# Autodesk Inventor assembly: Telemetry TAZ V1
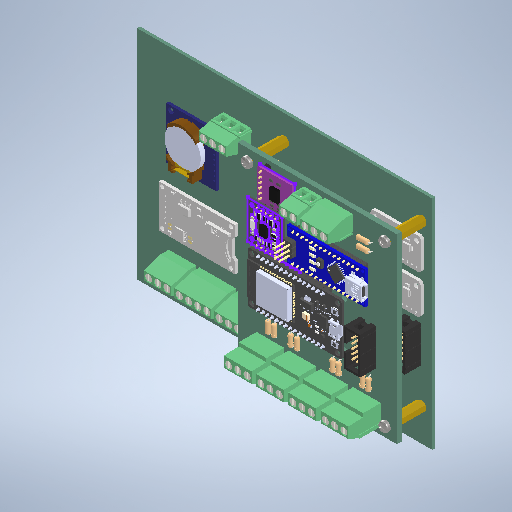
[picture p0: Inventor's stored thumbnail of the model, 512x512]
Saved by Autodesk Inventor 2025.2 (Build 292293000, 293)
## iProperties
Company: Kicad
Created: 2025-02-25
Part Number: Telemetry TAZ V1
Description: KiCad electronic assembly
Document SubType Name: Assembly
Designer: nugro
Authority: Unknown
Sending System: KiCad to STEP converter
Preprocessor: Open CASCADE STEP processor 7.8
Title: Telemetry TAZ V1.step
Author: Pcbnew
## Documents named in this file (9)
- C:\Users\nugro\Documents\KiCad\Telemetry TAZ V1\Telemetry TAZ V1\Telemetry TAZ V1\Telemetry TAZ V1\Telemetry TAZ V1.iam
- C:\Users\nugro\Documents\KiCad\Telemetry TAZ V1\Telemetry TAZ V1\Telemetry TAZ V1\Telemetry TAZ V1\TerminalBlock_Phoenix_MKDS-1,5-4-5.08_1x04_P5.08mm_Horizontal.iam
- C:\Users\nugro\Documents\KiCad\Telemetry TAZ V1\Telemetry TAZ V1\Telemetry TAZ V1\Telemetry TAZ V1\IDC-Header_2x05_P2.54mm_Vertical.iam
- C:\Users\nugro\Documents\KiCad\Telemetry TAZ V1\Telemetry TAZ V1\Telemetry TAZ V1\Telemetry TAZ V1\MicroSD Card Module - 2.iam
- C:\Users\nugro\Documents\KiCad\Telemetry TAZ V1\Telemetry TAZ V1\Telemetry TAZ V1\Telemetry TAZ V1\TerminalBlock_Phoenix_MKDS-1,5-3-5.08_1x03_P5.08mm_Horizontal.iam
- C:\Users\nugro\Documents\KiCad\Telemetry TAZ V1\Telemetry TAZ V1\Telemetry TAZ V1\Telemetry TAZ V1\16Bit I2C ADC+PGA - ADS1115.iam
- C:\Users\nugro\Documents\KiCad\Telemetry TAZ V1\Telemetry TAZ V1\Telemetry TAZ V1\Telemetry TAZ V1\HW-111_RTCmodule_DS1307.iam
- C:\Users\nugro\Documents\KiCad\Telemetry TAZ V1\Telemetry TAZ V1\Telemetry TAZ V1\Telemetry TAZ V1\Telemetry TAZ V1_PCB.ipt
- C:\Users\nugro\Documents\KiCad\IMU\IMU_1.5\IMU_1.5\IMU_1.5.iam
## Components (11 placed, 11 different names)
1. 4 [sub-assembly]
2. 6 [sub-assembly]
3. 8 [sub-assembly]
4. 10 [sub-assembly]
5. 12 [sub-assembly]
6. 13 [sub-assembly]
7. 15 [sub-assembly]
8. 16 [sub-assembly]
9. 17 [sub-assembly]
10. 18 — Mate:1
11. IMU_1.5:1 [sub-assembly] — Mate:1
## Relationships (1: Mate 1)
- Mate:1: 18 ↔ IMU_1.5:1
